# Autodesk Inventor assembly: SCR3D-6
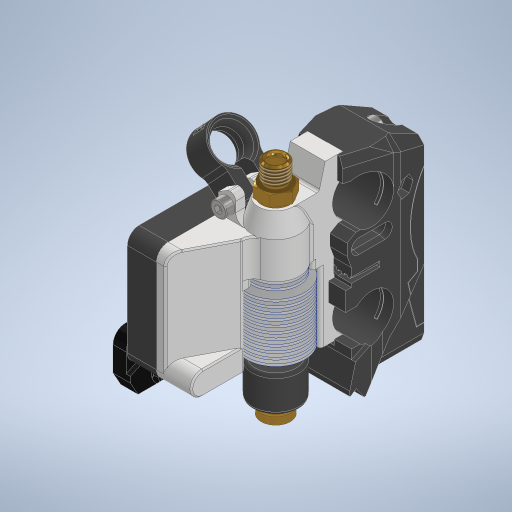
[picture p0: Inventor's stored thumbnail of the model, 512x512]
Saved by Autodesk Inventor 2023.1 (Build 271208000, 208)
## iProperties
Created: 2022-11-27
Part Number: SCR3D-6
Document SubType Name: Assembly
Designer: Frank
Author: Frank
## Documents named in this file (13)
- C:\Users\Frank\Desktop\SRC3D-6\SOURCE\SCR3D-6.iam
- C:\Users\Frank\Desktop\SRC3D-6\SOURCE\MINI-x-carriage.ipt
- C:\Users\Frank\Desktop\SRC3D-6\SOURCE\REVO-Micro Prusa Mini mount.ipt
- C:\Users\Frank\Desktop\SRC3D-6\SOURCE\Brass insert M3.ipt
- C:\Users\Frank\Desktop\SRC3D-6\SOURCE\REVO-Micro nozzle.ipt
- C:\Users\Frank\Desktop\SRC3D-6\SOURCE\REVO-Micro heatsink body.ipt
- C:\Users\Frank\Desktop\SRC3D-6\SOURCE\REVO-Micro heater body.ipt
- C:\Users\Frank\Desktop\SRC3D-6\SOURCE\MINI-male-threaded-fitting.ipt
- C:\Users\Frank\Desktop\SRC3D-6\SOURCE\MINI-fan-spacer-clip.ipt
- C:\Users\Frank\Desktop\SRC3D-6\SOURCE\MINI-extruder-fan-DS.ipt
- C:\Users\Frank\OneDrive\Documents\Inventor\Content Center Files\R2023\en-US\ISO 4762(2)\ISO 4762 - M3 x 20ISO.ipt
- C:\Users\Frank\OneDrive\Documents\Inventor\Content Center Files\R2023\en-US\ISO 4762(2)\ISO 4762 - M3 x 16ISO.ipt
- C:\Users\Frank\Desktop\SRC3D-6\SOURCE\MINI-minda-holder.ipt
## Components (19 placed, 12 different names)
1. MINI-x-carriage:1 — Mate:5, Mate:6, Mate:7, Mate:22, Mate:23, Mate:24, Mate:25, Mate:30
2. REVO-Micro Prusa Mini mount:1 — Mate:1, Mate:2, Mate:3, Mate:4, Flush:1, Flush:2, Flush:3, Flush:4, Flush:5, Flush:6, Angle:1, Angle:2, Mate:8, Mate:9, Flush:7, Flush:8, Mate:14, Mate:15, Flush:11, Mate:16, Mate:17, Mate:18, Mate:21, Mate:26, Mate:27
3. Brass insert M3:1 — Mate:1, Flush:1, Flush:5, Mate:5, Mate:7
4. Brass insert M3:2 — Mate:2, Flush:2, Flush:6, Mate:6
5. Brass insert M3:3 — Mate:3, Flush:3, Angle:1, Mate:19
6. Brass insert M3:4 — Mate:4, Flush:4, Angle:2, Mate:20
7. REVO-Micro heatsink body:1 — Mate:8, Mate:9, Mate:10, Mate:11, Flush:7, Flush:8, Flush:9
8. REVO-Micro nozzle:1 — Mate:10, Mate:11, Mate:12, Mate:13, Flush:9, Flush:10
9. REVO-Micro heater body:1 — Mate:12, Mate:13, Flush:10
10. MINI-male-threaded-fitting:1 — Mate:14, Mate:15, Flush:11
11. MINI-fan-spacer-clip:1 — Mate:16, Mate:17, Mate:18
12. MINI-extruder-fan-DS:1 — Mate:19, Mate:20, Mate:21, Mate:28, Mate:29, Mate:31, Mate:32
13. MINI-minda-holder:1 — Mate:30, Mate:31, Mate:32, Mate:33, Mate:34, Mate:35, Mate:36
14. ISO 4762 M3 x 20:1 — Mate:22, Mate:23
15. ISO 4762 M3 x 20:2 — Mate:24, Mate:25
16. ISO 4762 M3 x 20:3 — Mate:26, Mate:27
17. ISO 4762 M3 x 16:1 — Mate:28, Mate:29
18. ISO 4762 M3 x 16:2 — Mate:33, Mate:34
19. ISO 4762 M3 x 16:3 — Mate:35, Mate:36
## Relationships (49: Mate 36, Flush 11, Angle 2)
- Mate:1: REVO-Micro Prusa Mini mount:1 ↔ Brass insert M3:1
- Mate:2: REVO-Micro Prusa Mini mount:1 ↔ Brass insert M3:2
- Mate:3: REVO-Micro Prusa Mini mount:1 ↔ Brass insert M3:3
- Mate:4: REVO-Micro Prusa Mini mount:1 ↔ Brass insert M3:4
- Flush:1: REVO-Micro Prusa Mini mount:1 ↔ Brass insert M3:1
- Flush:2: REVO-Micro Prusa Mini mount:1 ↔ Brass insert M3:2
- Flush:3: REVO-Micro Prusa Mini mount:1 ↔ Brass insert M3:3
- Flush:4: REVO-Micro Prusa Mini mount:1 ↔ Brass insert M3:4
- Flush:5: REVO-Micro Prusa Mini mount:1 ↔ Brass insert M3:1
- Flush:6: REVO-Micro Prusa Mini mount:1 ↔ Brass insert M3:2
- Angle:1 (0 deg): REVO-Micro Prusa Mini mount:1 ↔ Brass insert M3:3
- Angle:2 (0 deg): REVO-Micro Prusa Mini mount:1 ↔ Brass insert M3:4
- Mate:5: MINI-x-carriage:1 ↔ Brass insert M3:1
- Mate:6: MINI-x-carriage:1 ↔ Brass insert M3:2
- Mate:7: MINI-x-carriage:1 ↔ Brass insert M3:1
- Mate:8: REVO-Micro Prusa Mini mount:1 ↔ REVO-Micro heatsink body:1
- Mate:9: REVO-Micro Prusa Mini mount:1 ↔ REVO-Micro heatsink body:1
- Mate:10: REVO-Micro heatsink body:1 ↔ REVO-Micro nozzle:1
- Mate:11: REVO-Micro heatsink body:1 ↔ REVO-Micro nozzle:1
- Mate:12: REVO-Micro nozzle:1 ↔ REVO-Micro heater body:1
- Mate:13: REVO-Micro nozzle:1 ↔ REVO-Micro heater body:1
- Flush:7: REVO-Micro Prusa Mini mount:1 ↔ REVO-Micro heatsink body:1
- Flush:8: REVO-Micro Prusa Mini mount:1 ↔ REVO-Micro heatsink body:1
- Flush:9: REVO-Micro heatsink body:1 ↔ REVO-Micro nozzle:1
- Flush:10: REVO-Micro nozzle:1 ↔ REVO-Micro heater body:1
- Mate:14: REVO-Micro Prusa Mini mount:1 ↔ MINI-male-threaded-fitting:1
- Mate:15: REVO-Micro Prusa Mini mount:1 ↔ MINI-male-threaded-fitting:1
- Flush:11: REVO-Micro Prusa Mini mount:1 ↔ MINI-male-threaded-fitting:1
- Mate:16: REVO-Micro Prusa Mini mount:1 ↔ MINI-fan-spacer-clip:1
- Mate:17: REVO-Micro Prusa Mini mount:1 ↔ MINI-fan-spacer-clip:1
- Mate:18: REVO-Micro Prusa Mini mount:1 ↔ MINI-fan-spacer-clip:1
- Mate:19: Brass insert M3:3 ↔ MINI-extruder-fan-DS:1
- Mate:20: Brass insert M3:4 ↔ MINI-extruder-fan-DS:1
- Mate:21: REVO-Micro Prusa Mini mount:1 ↔ MINI-extruder-fan-DS:1
- Mate:22: MINI-x-carriage:1 ↔ ISO 4762 M3 x 20:1
- Mate:23: MINI-x-carriage:1 ↔ ISO 4762 M3 x 20:1
- Mate:24: MINI-x-carriage:1 ↔ ISO 4762 M3 x 20:2
- Mate:25: MINI-x-carriage:1 ↔ ISO 4762 M3 x 20:2
- Mate:26: REVO-Micro Prusa Mini mount:1 ↔ ISO 4762 M3 x 20:3
- Mate:27: REVO-Micro Prusa Mini mount:1 ↔ ISO 4762 M3 x 20:3
- Mate:28: MINI-extruder-fan-DS:1 ↔ ISO 4762 M3 x 16:1
- Mate:29: MINI-extruder-fan-DS:1 ↔ ISO 4762 M3 x 16:1
- Mate:30: MINI-x-carriage:1 ↔ MINI-minda-holder:1
- Mate:31: MINI-extruder-fan-DS:1 ↔ MINI-minda-holder:1
- Mate:32: MINI-extruder-fan-DS:1 ↔ MINI-minda-holder:1
- Mate:33: MINI-minda-holder:1 ↔ ISO 4762 M3 x 16:2
- Mate:34: MINI-minda-holder:1 ↔ ISO 4762 M3 x 16:2
- Mate:35: MINI-minda-holder:1 ↔ ISO 4762 M3 x 16:3
- Mate:36: MINI-minda-holder:1 ↔ ISO 4762 M3 x 16:3
